# Autodesk Inventor assembly: Сборка8
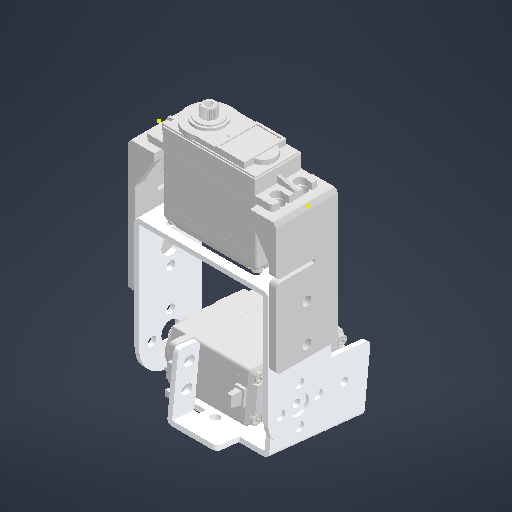
[picture p0: Inventor's stored thumbnail of the model, 512x512]
Saved by Autodesk Inventor 2025 (Build 290162000, 162)
## iProperties
Created: 2025-02-15
Part Number: Сборка8
Document SubType Name: Assembly
Designer: Phantom
Author: Phantom
## Documents named in this file (5)
- C:\Users\Phantom\Desktop\Phantom16950\Сборка8.iam
- C:\Users\Phantom\Downloads\39593_txm-standard-scale pivot armwbearing\39593_txm-standard-scale pivot armwbearing.ipt
- C:\Users\Phantom\Desktop\Phantom16950\2000-0025-0002\2000-0025-0002_MIR4_MIR1_MIR.ipt
- C:\Users\Phantom\Desktop\Phantom16950\для захвата.ipt
- C:\Users\Phantom\Desktop\Phantom16950\39060_txm-standard servo bracket\39060_txm-standard servo bracket_MIR1.ipt
## Components (6 placed, 4 different names)
1. 39593_txm-standard-scale pivot armwbearing:1 — Совмещение:1, Совмещение:2, Совмещение:3, Совмещение:4, Заподлицо:1, Совмещение:6, Совмещение:7
2. 2000-0025-0002_MIR4_MIR1_MIR:1 — Совмещение:1, Совмещение:2
3. для захвата:1 — Совмещение:3, Совмещение:4, Совмещение:5
4. для захвата:2 — Заподлицо:1, Совмещение:5, Совмещение:6
5. 39060_txm-standard servo bracket_MIR1:1 — Совмещение:7, Совмещение:8, Совмещение:9
6. 2000-0025-0002_MIR4_MIR1_MIR:2 — Совмещение:8, Совмещение:9
## Relationships (10: Mate 9, Flush 1)
- Совмещение:1 [Mate]: 39593_txm-standard-scale pivot armwbearing:1 ↔ 2000-0025-0002_MIR4_MIR1_MIR:1
- Совмещение:2 [Mate]: 39593_txm-standard-scale pivot armwbearing:1 ↔ 2000-0025-0002_MIR4_MIR1_MIR:1
- Совмещение:3 [Mate]: 39593_txm-standard-scale pivot armwbearing:1 ↔ для захвата:1
- Совмещение:4 [Mate]: 39593_txm-standard-scale pivot armwbearing:1 ↔ для захвата:1
- Заподлицо:1 [Flush]: 39593_txm-standard-scale pivot armwbearing:1 ↔ для захвата:2
- Совмещение:5 [Mate]: для захвата:1 ↔ для захвата:2
- Совмещение:6 [Mate]: 39593_txm-standard-scale pivot armwbearing:1 ↔ для захвата:2
- Совмещение:7 [Mate]: 39593_txm-standard-scale pivot armwbearing:1 ↔ 39060_txm-standard servo bracket_MIR1:1
- Совмещение:8 [Mate]: 39060_txm-standard servo bracket_MIR1:1 ↔ 2000-0025-0002_MIR4_MIR1_MIR:2
- Совмещение:9 [Mate]: 39060_txm-standard servo bracket_MIR1:1 ↔ 2000-0025-0002_MIR4_MIR1_MIR:2
